# Autodesk Inventor assembly: gusset_frame
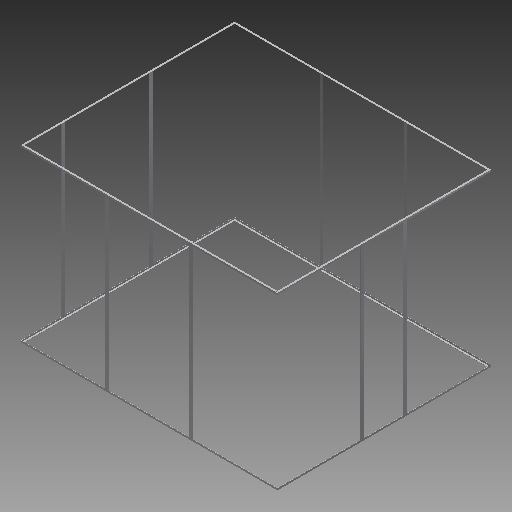
[picture p0: Inventor's stored thumbnail of the model, 512x512]
Saved by Autodesk Inventor 2019 (Build 230136000, 136)
## iProperties
Created: 2018-07-11
Part Number: gusset_frame
Document SubType Name: Assembly
Designer: User
Author: User
## Documents named in this file (4)
- C:\Users\User\Documents\GitHub\darkRadio\3D Models\Room Model\gusset_frame.iam
- C:\Users\User\Documents\GitHub\darkRadio\3D Models\Room Model\gusset_roofFloor.iam
- C:\Users\User\Documents\GitHub\darkRadio\3D Models\Room Model\gusset_plate.ipt
- C:\Users\User\Documents\GitHub\darkRadio\3D Models\Room Model\params.xlsx
## Components (10 placed, 2 different names)
1. gusset_roofFloor:1 [sub-assembly] — Mate:1, Flush:1, Mate:2, Flush:2, Mate:3, Flush:3, Mate:4, Flush:4, Mate:5, Flush:5, Mate:6, Flush:6, Mate:7, Flush:7, Mate:8, Flush:8, Flush:11, Flush:13, Mate:11, Mate:16
2. gusset_plate:1 — Mate:1, Flush:1, Mate:16, Mate:12
3. gusset_plate:2 — Mate:2, Flush:2, Flush:10, Mate:12
4. gusset_plate:3 — Mate:3, Flush:3, Mate:9, Flush:9, Flush:11, Flush:12
5. gusset_plate:4 — Mate:4, Flush:4, Flush:12
6. gusset_plate:5 — Mate:5, Flush:5, Flush:13, Mate:10
7. gusset_plate:6 — Mate:6, Flush:6, Mate:10
8. gusset_plate:7 — Mate:7, Flush:7, Mate:11, Flush:14
9. gusset_plate:8 — Mate:8, Flush:8, Flush:14
10. gusset_roofFloor:2 [sub-assembly] — Mate:9, Flush:9, Flush:10
## Relationships (27: Flush 14, Mate 13)
- Mate:1: gusset_roofFloor:1 ↔ gusset_plate:1
- Flush:1: gusset_roofFloor:1 ↔ gusset_plate:1
- Mate:2: gusset_roofFloor:1 ↔ gusset_plate:2
- Flush:2: gusset_roofFloor:1 ↔ gusset_plate:2
- Mate:3: gusset_roofFloor:1 ↔ gusset_plate:3
- Flush:3: gusset_roofFloor:1 ↔ gusset_plate:3
- Mate:4: gusset_roofFloor:1 ↔ gusset_plate:4
- Flush:4: gusset_roofFloor:1 ↔ gusset_plate:4
- Mate:5: gusset_roofFloor:1 ↔ gusset_plate:5
- Flush:5: gusset_roofFloor:1 ↔ gusset_plate:5
- Mate:6: gusset_roofFloor:1 ↔ gusset_plate:6
- Flush:6: gusset_roofFloor:1 ↔ gusset_plate:6
- Mate:7: gusset_roofFloor:1 ↔ gusset_plate:7
- Flush:7: gusset_roofFloor:1 ↔ gusset_plate:7
- Mate:8: gusset_roofFloor:1 ↔ gusset_plate:8
- Flush:8: gusset_roofFloor:1 ↔ gusset_plate:8
- Mate:9: gusset_plate:3 ↔ gusset_roofFloor:2
- Flush:9: gusset_plate:3 ↔ gusset_roofFloor:2
- Flush:10: gusset_plate:2 ↔ gusset_roofFloor:2
- Flush:11 (1216.025 mm): gusset_roofFloor:1 ↔ gusset_plate:3
- Flush:12 (1196.975 mm): gusset_plate:3 ↔ gusset_plate:4
- Flush:13 (1200.15 mm): gusset_roofFloor:1 ↔ gusset_plate:5
- Mate:10 (-660.4 mm): gusset_plate:5 ↔ gusset_plate:6
- Mate:11 (-1257.3 mm): gusset_roofFloor:1 ↔ gusset_plate:7
- Flush:14 (1200.15 mm): gusset_plate:7 ↔ gusset_plate:8
- Mate:16 (-628.65 mm): gusset_roofFloor:1 ↔ gusset_plate:1
- Mate:12 (1200.15 mm): gusset_plate:1 ↔ gusset_plate:2
## Named parameters: wallThick = 44.45 mm, roomWidth = 3048 mm, roomDepth = 3657.6 mm, roomHeight = 2438.4 mm, doorWidth = 895.35 mm, doorHeight = 2108.2 mm, doorX = 774.7 mm, doorY = 88.9 mm, doorLip = 76.2 mm, doorThick = 57.15 mm, tubeD = 19.05 mm, tubeTurnR = 76.2 mm
